# Autodesk Inventor assembly: Modbay
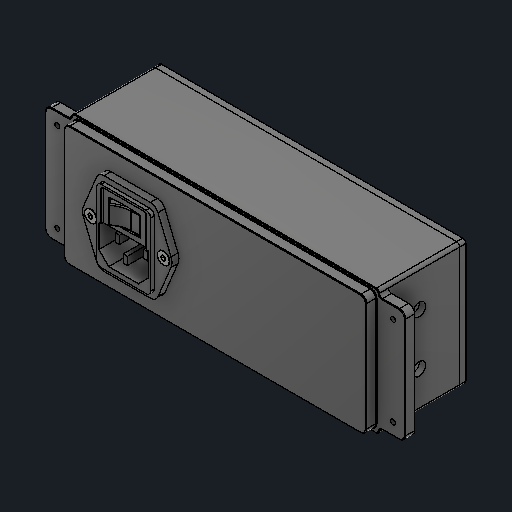
[picture p0: Inventor's stored thumbnail of the model, 512x512]
Saved by Autodesk Inventor 2026.2 (Build 302298000, 298)
## iProperties
Created: 2026-08-18
Part Number: Modbay
Document SubType Name: Assembly
Designer: JoshuaEah
Author: JoshuaEah
## Documents named in this file (5)
- C:\Users\JoshuaEah\Documents\GitHub\Designed-Trinkets\Guitar\Modular Pedalboard\Modbay.iam
- C:\Users\JoshuaEah\Documents\GitHub\Designed-Trinkets\Guitar\Modular Pedalboard\Junction Box Modbay.ipt
- C:\Users\JoshuaEah\Documents\GitHub\Designed-Trinkets\Guitar\Modular Pedalboard\Hardware\C14 Inlet.ipt
- C:\Users\JoshuaEah\Documents\GitHub\Designed-Trinkets\Guitar\Modular Pedalboard\Junction Box Modbay Cover.ipt
- C:\Users\JoshuaEah\Documents\GitHub\Designed-Trinkets\Guitar\Modular Pedalboard\Hardware\Fasteners\M3x10 FHCS.ipt
## Components (5 placed, 4 different names)
1. Junction Box Modbay:1 — Insert:1, Insert:2
2. C14 Inlet:1 — Insert:1, Insert:3, Insert:4
3. M3x10 FHCS:1 — Insert:3
4. M3x10 FHCS:2 — Insert:4
5. Junction Box Modbay Cover:1 — Insert:2
## Relationships (4: Insert 4)
- Insert:1: Junction Box Modbay:1 ↔ C14 Inlet:1
- Insert:3: C14 Inlet:1 ↔ M3x10 FHCS:1
- Insert:4: C14 Inlet:1 ↔ M3x10 FHCS:2
- Insert:2: Junction Box Modbay:1 ↔ Junction Box Modbay Cover:1
